# Autodesk Inventor assembly: Piston Subassembly
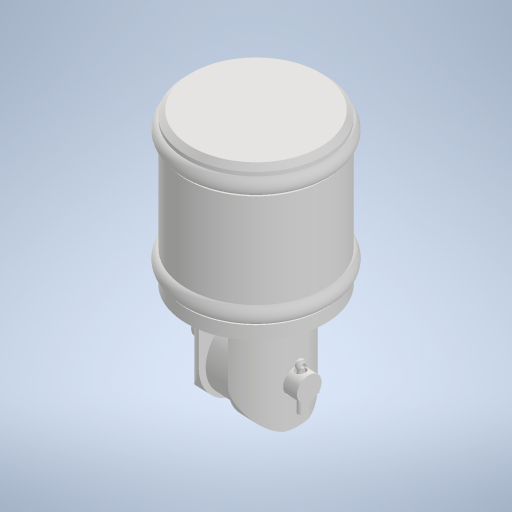
[picture p0: Inventor's stored thumbnail of the model, 512x512]
Saved by Autodesk Inventor 2023 (Build 270158000, 158)
## iProperties
Created: 2022-12-22
Part Number: Piston Subassembly
Document SubType Name: Assembly
Designer: tgr41
Author: tgr41
## Documents named in this file (6)
- C:\Users\tgr41\OneDrive\Documents\Repositories\Steam-Engine\1.5x1 Inch 3 Cylidner\Cast Engine Block Design V4\A.Piston Subassembly.iam
- C:\Users\tgr41\OneDrive\Documents\Repositories\Steam-Engine\1.5x1 Inch 3 Cylidner\Cast Engine Block Design V4\P.Piston.ipt
- C:\Users\tgr41\OneDrive\Documents\Repositories\Steam-Engine\1.5x1 Inch 3 Cylidner\Cast Engine Block Design V4\P.Wrist Pin.ipt
- C:\Users\tgr41\OneDrive\Documents\Repositories\Steam-Engine\1.5x1 Inch 3 Cylidner\Cast Engine Block Design V4\P.Cotter Pin.ipt
- C:\Users\tgr41\OneDrive\Documents\Repositories\Steam-Engine\1.5x1 Inch 3 Cylidner\Cast Engine Block Design V4\P.Piston O Ring.ipt
- C:\Users\tgr41\OneDrive\Documents\Repositories\Steam-Engine\1.5x1 Inch 3 Cylidner\Cast Engine Block Design V4\P.Wrist Pin Bearing.ipt
## Components (7 placed, 5 different names)
1. P.Piston:1 — Mate:1, Tangent:2, Angle:1, Angle:2, Angle:3, Angle:4, Mate:5, Tangent:4, Tangent:5, Mate:6, Mate:7
2. P.Wrist Pin:1 — Mate:1, Mate:2, Tangent:1, Tangent:2, Mate:3, Tangent:3, Mate:4
3. P.Cotter Pin:1 — Mate:3, Tangent:3, Angle:2, Angle:4
4. P.Cotter Pin:2 — Mate:2, Tangent:1, Angle:1, Angle:3
5. P.Piston O Ring:1 — Tangent:5, Mate:6
6. P.Wrist Pin Bearing:1 — Mate:4, Mate:5
7. P.Piston O Ring:2 — Tangent:4, Mate:7
## Relationships (16: Mate 7, Tangent 5, Angle 4)
- Mate:1: P.Piston:1 ↔ P.Wrist Pin:1
- Mate:2: P.Wrist Pin:1 ↔ P.Cotter Pin:2
- Tangent:1: P.Wrist Pin:1 ↔ P.Cotter Pin:2
- Tangent:2: P.Piston:1 ↔ P.Wrist Pin:1
- Angle:1 (90 deg): P.Piston:1 ↔ P.Cotter Pin:2
- Mate:3: P.Wrist Pin:1 ↔ P.Cotter Pin:1
- Tangent:3: P.Wrist Pin:1 ↔ P.Cotter Pin:1
- Angle:2 (-90 deg): P.Piston:1 ↔ P.Cotter Pin:1
- Angle:3 (180 deg): P.Piston:1 ↔ P.Cotter Pin:2
- Angle:4 (0 deg): P.Piston:1 ↔ P.Cotter Pin:1
- Mate:4: P.Wrist Pin:1 ↔ P.Wrist Pin Bearing:1
- Mate:5: P.Piston:1 ↔ P.Wrist Pin Bearing:1
- Tangent:4: P.Piston:1 ↔ P.Piston O Ring:2
- Tangent:5: P.Piston:1 ↔ P.Piston O Ring:1
- Mate:6: P.Piston:1 ↔ P.Piston O Ring:1
- Mate:7: P.Piston:1 ↔ P.Piston O Ring:2
